# Autodesk Inventor assembly: platform
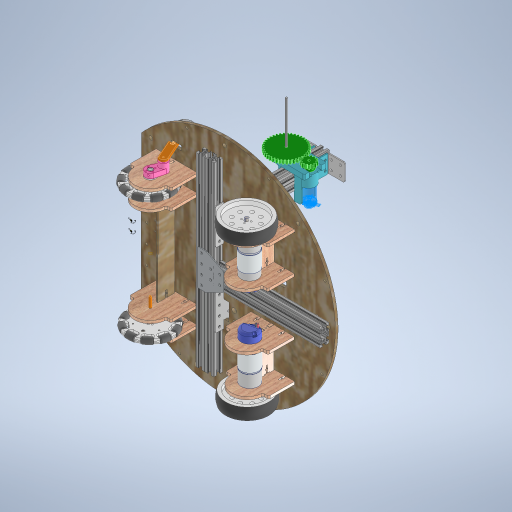
[picture p0: Inventor's stored thumbnail of the model, 512x512]
Saved by Autodesk Inventor 2023.1 (Build 271208000, 208)
## iProperties
Created: 2023-03-13
Part Number: platform
Document SubType Name: Assembly
Designer: User
Author: User
## Documents named in this file (48)
- C:\Users\DELL\reposGitHub\Cheburashka\Cheburashka_construction\platform\platform.iam
- C:\Users\DELL\reposGitHub\Cheburashka\Cheburashka_construction\platform\Osn. platform.ipt
- C:\Users\DELL\reposGitHub\Cheburashka\Cheburashka_construction\platform\motor1.ipt
- C:\Users\DELL\reposGitHub\Cheburashka\Cheburashka_construction\platform\motor2.ipt
- C:\Users\DELL\reposGitHub\Cheburashka\Cheburashka_construction\platform\motor3.ipt
- C:\Users\DELL\reposGitHub\Cheburashka\Cheburashka_construction\platform\wheel1.ipt
- C:\Users\DELL\reposGitHub\Cheburashka\Cheburashka_construction\platform\44260_txm torquenado dc motor_MIR2.ipt
- C:\Users\DELL\reposGitHub\Cheburashka\Cheburashka_construction\platform\36466_txm-4 inch omni wheel.ipt
- C:\Users\DELL\reposGitHub\Cheburashka\Cheburashka_construction\platform\39055_txm-4 inch wheel_MIR1.ipt
- C:\Users\DELL\reposGitHub\Cheburashka\Cheburashka_construction\platform\motor1_MIR3.ipt
- C:\Users\DELL\reposGitHub\Cheburashka\Cheburashka_construction\platform\motor2_MIR3.ipt
- C:\Users\DELL\reposGitHub\Cheburashka\Cheburashka_construction\platform\motor3_MIR3.ipt
- C:\Users\DELL\reposGitHub\Cheburashka\Cheburashka_construction\platform\44260_txm torquenado dc motor_MIR2_MIR.ipt
- C:\Users\DELL\reposGitHub\Cheburashka\Cheburashka_construction\platform\wheel1_MIR.ipt
- C:\Users\DELL\reposGitHub\Cheburashka\Cheburashka_construction\platform\36466_txm-4 inch omni wheel_MIR2.ipt
- C:\Users\DELL\reposGitHub\Cheburashka\Cheburashka_construction\platform\39055_txm-4 inch wheel_MIR1_MIR.ipt
- C:\Users\DELL\reposGitHub\Cheburashka\Cheburashka_construction\platform\кривошип.ipt
- C:\Users\DELL\reposGitHub\Cheburashka\Cheburashka_construction\platform\ось колес2.ipt
- C:\Users\DELL\reposGitHub\Cheburashka\Cheburashka_construction\platform\akfytw2.ipt
- C:\Users\DELL\reposGitHub\Cheburashka\Cheburashka_construction\platform\подшипник2.ipt
- C:\Users\DELL\reposGitHub\Cheburashka\Cheburashka_construction\platform\шатун22.ipt
- C:\Users\DELL\reposGitHub\Cheburashka\Cheburashka_construction\platform\обр_профиль.ipt
- C:\Users\DELL\reposGitHub\Cheburashka\Cheburashka_construction\platform\обр_профиль2.ipt
- C:\Users\DELL\reposGitHub\Cheburashka\Cheburashka_construction\platform\8bc17c1464c21f56fb2a3979b7c6b729.ipt
- C:\Users\DELL\reposGitHub\Cheburashka\Cheburashka_construction\platform\L72-T_soedinitel-60kh80.ipt
- C:\Users\DELL\reposGitHub\Cheburashka\Cheburashka_construction\platform\ребро.ipt
- C:\Users\DELL\reposGitHub\Cheburashka\Cheburashka_construction\platform\стенд.ipt
- C:\Users\DELL\reposGitHub\Cheburashka\Cheburashka_construction\platform\Raspberry Pi Camera Stand - 274111\files\camera_back_cover_v002.ipt
- C:\Users\DELL\reposGitHub\Cheburashka\Cheburashka_construction\platform\Raspberry Pi Camera Stand - 274111\files\camera_front_box_v003.ipt
- C:\Users\DELL\reposGitHub\Cheburashka\Cheburashka_construction\platform\4ad8d019baf454c6bbd45c2c6ffb6783.ipt
- C:\Users\DELL\reposGitHub\Cheburashka\Cheburashka_construction\platform\гриб.ipt
- C:\Users\DELL\reposGitHub\Cheburashka\Cheburashka_construction\platform\legs\myMotorHolder.ipt
- C:\Users\DELL\reposGitHub\Cheburashka\Cheburashka_construction\platform\legs\myBering.ipt
- C:\Users\DELL\reposGitHub\Cheburashka\Cheburashka_construction\platform\legs\POLULU final.ipt
- C:\Users\DELL\reposGitHub\Cheburashka\Cheburashka_construction\platform\legs\axis.ipt
- C:\Users\DELL\reposGitHub\Cheburashka\Cheburashka_construction\platform\legs\bering.ipt
- C:\Users\DELL\reposGitHub\Cheburashka\Cheburashka_construction\platform\8bc17c1464c21f56fb2a3979b7c6b729_MIR.ipt
- C:\Users\DELL\reposGitHub\Cheburashka\Cheburashka_construction\platform\legs\myMotorHolder_MIR.ipt
- C:\Users\DELL\reposGitHub\Cheburashka\Cheburashka_construction\platform\legs\POLULU final_MIR.ipt
- C:\Users\DELL\reposGitHub\Cheburashka\Cheburashka_construction\platform\legs\myBering_MIR.ipt
- C:\Users\DELL\reposGitHub\Cheburashka\Cheburashka_construction\platform\legs\axis_MIR.ipt
- C:\Users\DELL\reposGitHub\Cheburashka\Cheburashka_construction\platform\legs\bering_MIR.ipt
- C:\Users\DELL\reposGitHub\Cheburashka\Cheburashka_construction\platform\legs\шестерня12 (2).ipt
- C:\Users\DELL\reposGitHub\Cheburashka\Cheburashka_construction\platform\legs\шестерня36_v2.ipt
- C:\Users\DELL\reposGitHub\Cheburashka\Cheburashka_construction\platform\legs\шестерня12 (2)_MIR.ipt
- C:\Users\DELL\reposGitHub\Cheburashka\Cheburashka_construction\platform\legs\шестерня36_v2_MIR.ipt
- C:\Users\DELL\reposGitHub\Cheburashka\Cheburashka_construction\platform\8bc17c1464c21f56fb2a3979b7c6b729_MIR1.ipt
- C:\Users\DELL\reposGitHub\Cheburashka\Cheburashka_construction\platform\подш_ноги.ipt
## Components (60 placed, 47 different names)
1. Osn. platform:1 — Совмещение:129, Совмещение:130, Совмещение:131, Совмещение:132, Совмещение:133, Совмещение:137, Совмещение:138, Совмещение:155, Совмещение:158, Совмещение:178, Совмещение:181, Совмещение:182, Совмещение:183, Совмещение:184, Совмещение:185, Совмещение:186, Совмещение:192, Совмещение:193, Совмещение:194, Совмещение:195, Совмещение:196, Совмещение:197, Совмещение:198, Совмещение:217, Совмещение:218, Совмещение:219, Совмещение:230, Совмещение:231, Совмещение:232, Совмещение:233, Совмещение:280, Совмещение:281, Совмещение:282
2. motor1:1 — Совмещение:181, Совмещение:182
3. motor2:1 — Совмещение:232, Совмещение:233
4. motor3:1 — Совмещение:230, Совмещение:231
5. 44260_txm torquenado dc motor_MIR2:1 — Совмещение:21
6. wheel1:1 — Совмещение:101, Совмещение:185, Совмещение:186
7. 36466_txm-4 inch omni wheel:1
8. 39055_txm-4 inch wheel_MIR1:1 — Совмещение:21
9. motor1_MIR3:1 — Совмещение:183, Совмещение:184
10. motor2_MIR3:1 — Совмещение:148
11. motor3_MIR3:1 — Совмещение:109, Совмещение:110, Совмещение:111
12. 44260_txm torquenado dc motor_MIR2_MIR:1 — Совмещение:28, Совмещение:109, Совмещение:110, Совмещение:148
13. wheel1_MIR:1 — Совмещение:192, Совмещение:197, Совмещение:198, Совмещение:228
14. wheel1_MIR:2 — Совмещение:195, Совмещение:196
15. 36466_txm-4 inch omni wheel_MIR2:1 — Совмещение:229
16. 39055_txm-4 inch wheel_MIR1_MIR:1 — Совмещение:28, Совмещение:111
17. кривошип:1 — Совмещение:90, Совмещение:91, Совмещение:92, Совмещение:93, Совмещение:96
18. ось колес2:1 — Совмещение:228, Совмещение:229, Совмещение:283
19. akfytw2:1 — Совмещение:90, Совмещение:91, Совмещение:101, Совмещение:283
20. подшипник2:1 — Совмещение:92, Совмещение:93, Совмещение:94
21. подшипник2:2 — Совмещение:94, Совмещение:95
22. шатун22:1 — Совмещение:95, Совмещение:96, Совмещение:225, Совмещение:226, Совмещение:227
23. обр_профиль:1 — Совмещение:129, Совмещение:130, Совмещение:131, Совмещение:179, Совмещение:206, Совмещение:207, Совмещение:208, Совмещение:210, Симметрия:1
24. обр_профиль:2 — Совмещение:132, Совмещение:133, Совмещение:135, Совмещение:136, Совмещение:157, Совмещение:212, Совмещение:237, Совмещение:238, Совмещение:242, Совмещение:243, Совмещение:250, Совмещение:252, Совмещение:253, Заподлицо:1, Заподлицо:2, Симметрия:1, Совмещение:290
25. обр_профиль2:1 — Совмещение:135, Совмещение:136, Совмещение:139, Совмещение:204, Совмещение:205, Совмещение:209, Совмещение:211
26. обр_профиль:3 — Совмещение:137, Совмещение:138, Совмещение:139
27. 8bc17c1464c21f56fb2a3979b7c6b729:1 — Совмещение:155, Совмещение:206, Совмещение:207
28. 8bc17c1464c21f56fb2a3979b7c6b729:2 — Совмещение:157, Совмещение:158
29. L72-T_soedinitel-60kh80:1 — Совмещение:209, Совмещение:210
30. L72-T_soedinitel-60kh80:2 — Совмещение:211, Совмещение:212
31. L72-T_soedinitel-60kh80:3 — Совмещение:204, Совмещение:205
32. ребро:1 — Совмещение:201, Совмещение:202, Совмещение:203
33. camera_back_cover_v002:1 — Совмещение:222, Совмещение:223, Совмещение:224
34. camera_front_box_v003:1 — Совмещение:220, Совмещение:221, Совмещение:222, Совмещение:223, Совмещение:224
35. 4ad8d019baf454c6bbd45c2c6ffb6783:1 — Совмещение:178, Совмещение:179, Совмещение:208
36. wheel1:2 — Совмещение:193, Совмещение:194, Совмещение:201, Совмещение:202, Совмещение:203
37. стенд:1 — Совмещение:217, Совмещение:218, Совмещение:219, Совмещение:220, Совмещение:221
38. гриб:1 — Совмещение:225, Совмещение:226, Совмещение:227
39. 8bc17c1464c21f56fb2a3979b7c6b729:3 — Совмещение:237, Совмещение:238, Заподлицо:2, Совмещение:291
40. myMotorHolder:1 — Совмещение:247, Совмещение:270, Заподлицо:4, Совмещение:286, Совмещение:289, Совмещение:290, Совмещение:291
41. 8bc17c1464c21f56fb2a3979b7c6b729:4 — Совмещение:242, Совмещение:243, Совмещение:251, Заподлицо:1
42. myBering:1 — Совмещение:250, Совмещение:251, Совмещение:252, Совмещение:253, Совмещение:259
43. POLULU final:1 — Совмещение:247, Совмещение:269
44. axis:1 — Совмещение:287
45. bering:1 — Совмещение:289
46. bering:2 — Совмещение:259
47. 8bc17c1464c21f56fb2a3979b7c6b729_MIR:1 — Совмещение:277, Совмещение:278, Совмещение:279
48. myMotorHolder_MIR:1 — Совмещение:262, Совмещение:263, Совмещение:277, Совмещение:278, Совмещение:279
49. POLULU final_MIR:1 — Совмещение:262, Совмещение:263
50. myBering_MIR:1 — Совмещение:264, Совмещение:265, Совмещение:266, Совмещение:267
51. axis_MIR:1 — Совмещение:264, Совмещение:268
52. bering_MIR:1 — Совмещение:265, Совмещение:266
53. bering_MIR:2 — Совмещение:267, Совмещение:268
54. шестерня12 (2):1 — Совмещение:269, Совмещение:270
55. шестерня36_v2:1 — Совмещение:285, Совмещение:286, Совмещение:287
56. 4ad8d019baf454c6bbd45c2c6ffb6783:2 — Совмещение:280, Совмещение:281, Совмещение:282
57. шестерня12 (2)_MIR:1
58. шестерня36_v2_MIR:1
59. 8bc17c1464c21f56fb2a3979b7c6b729_MIR1:1
60. подш_ноги:1 — Заподлицо:4, Совмещение:285
## Relationships (107: Mate 103, Flush 3, Symmetry 1)
- Совмещение:21 [Mate]: 44260_txm torquenado dc motor_MIR2:1 ↔ 39055_txm-4 inch wheel_MIR1:1
- Совмещение:28 [Mate]: 44260_txm torquenado dc motor_MIR2_MIR:1 ↔ 39055_txm-4 inch wheel_MIR1_MIR:1
- Совмещение:90 [Mate]: кривошип:1 ↔ akfytw2:1
- Совмещение:91 [Mate]: кривошип:1 ↔ akfytw2:1
- Совмещение:92 [Mate]: кривошип:1 ↔ подшипник2:1
- Совмещение:93 [Mate]: кривошип:1 ↔ подшипник2:1
- Совмещение:94 [Mate]: подшипник2:1 ↔ подшипник2:2
- Совмещение:95 [Mate]: подшипник2:2 ↔ шатун22:1
- Совмещение:96 [Mate] (2 mm): кривошип:1 ↔ шатун22:1
- Совмещение:101 [Mate]: wheel1:1 ↔ akfytw2:1
- Совмещение:109 [Mate]: motor3_MIR3:1 ↔ 44260_txm torquenado dc motor_MIR2_MIR:1
- Совмещение:110 [Mate]: motor3_MIR3:1 ↔ 44260_txm torquenado dc motor_MIR2_MIR:1
- Совмещение:111 [Mate] (5 mm): motor3_MIR3:1 ↔ 39055_txm-4 inch wheel_MIR1_MIR:1
- Совмещение:129 [Mate]: Osn. platform:1 ↔ обр_профиль:1
- Совмещение:130 [Mate]: Osn. platform:1 ↔ обр_профиль:1
- Совмещение:131 [Mate]: Osn. platform:1 ↔ обр_профиль:1
- Совмещение:132 [Mate]: Osn. platform:1 ↔ обр_профиль:2
- Совмещение:133 [Mate]: Osn. platform:1 ↔ обр_профиль:2
- Совмещение:135 [Mate] (99.253 mm): обр_профиль:2 ↔ обр_профиль2:1
- Совмещение:136 [Mate]: обр_профиль:2 ↔ обр_профиль2:1
- Совмещение:137 [Mate]: Osn. platform:1 ↔ обр_профиль:3
- Совмещение:138 [Mate] (4.43 mm): Osn. platform:1 ↔ обр_профиль:3
- Совмещение:139 [Mate]: обр_профиль2:1 ↔ обр_профиль:3
- Совмещение:148 [Mate]: motor2_MIR3:1 ↔ 44260_txm torquenado dc motor_MIR2_MIR:1
- Совмещение:155 [Mate]: Osn. platform:1 ↔ 8bc17c1464c21f56fb2a3979b7c6b729:1
- Совмещение:157 [Mate]: обр_профиль:2 ↔ 8bc17c1464c21f56fb2a3979b7c6b729:2
- Совмещение:158 [Mate]: Osn. platform:1 ↔ 8bc17c1464c21f56fb2a3979b7c6b729:2
- Совмещение:178 [Mate]: Osn. platform:1 ↔ 4ad8d019baf454c6bbd45c2c6ffb6783:1
- Совмещение:179 [Mate]: обр_профиль:1 ↔ 4ad8d019baf454c6bbd45c2c6ffb6783:1
- Совмещение:181 [Mate]: Osn. platform:1 ↔ motor1:1
- Совмещение:182 [Mate]: Osn. platform:1 ↔ motor1:1
- Совмещение:183 [Mate]: Osn. platform:1 ↔ motor1_MIR3:1
- Совмещение:184 [Mate]: Osn. platform:1 ↔ motor1_MIR3:1
- Совмещение:185 [Mate]: Osn. platform:1 ↔ wheel1:1
- Совмещение:186 [Mate]: Osn. platform:1 ↔ wheel1:1
- Совмещение:192 [Mate]: Osn. platform:1 ↔ wheel1_MIR:1
- Совмещение:193 [Mate]: Osn. platform:1 ↔ wheel1:2
- Совмещение:194 [Mate]: Osn. platform:1 ↔ wheel1:2
- Совмещение:195 [Mate]: Osn. platform:1 ↔ wheel1_MIR:2
- Совмещение:196 [Mate]: Osn. platform:1 ↔ wheel1_MIR:2
- Совмещение:197 [Mate]: Osn. platform:1 ↔ wheel1_MIR:1
- Совмещение:198 [Mate]: Osn. platform:1 ↔ wheel1_MIR:1
- Совмещение:201 [Mate]: ребро:1 ↔ wheel1:2
- Совмещение:202 [Mate]: ребро:1 ↔ wheel1:2
- Совмещение:203 [Mate]: ребро:1 ↔ wheel1:2
- Совмещение:204 [Mate]: обр_профиль2:1 ↔ L72-T_soedinitel-60kh80:3
- Совмещение:205 [Mate]: обр_профиль2:1 ↔ L72-T_soedinitel-60kh80:3
- Совмещение:206 [Mate]: обр_профиль:1 ↔ 8bc17c1464c21f56fb2a3979b7c6b729:1
- Совмещение:207 [Mate]: обр_профиль:1 ↔ 8bc17c1464c21f56fb2a3979b7c6b729:1
- Совмещение:208 [Mate]: обр_профиль:1 ↔ 4ad8d019baf454c6bbd45c2c6ffb6783:1
- Совмещение:209 [Mate]: обр_профиль2:1 ↔ L72-T_soedinitel-60kh80:1
- Совмещение:210 [Mate]: обр_профиль:1 ↔ L72-T_soedinitel-60kh80:1
- Совмещение:211 [Mate]: обр_профиль2:1 ↔ L72-T_soedinitel-60kh80:2
- Совмещение:212 [Mate]: обр_профиль:2 ↔ L72-T_soedinitel-60kh80:2
- Совмещение:217 [Mate]: Osn. platform:1 ↔ стенд:1
- Совмещение:218 [Mate]: Osn. platform:1 ↔ стенд:1
- Совмещение:219 [Mate]: Osn. platform:1 ↔ стенд:1
- Совмещение:220 [Mate]: camera_front_box_v003:1 ↔ стенд:1
- Совмещение:221 [Mate]: camera_front_box_v003:1 ↔ стенд:1
- Совмещение:222 [Mate]: camera_back_cover_v002:1 ↔ camera_front_box_v003:1
- Совмещение:223 [Mate]: camera_back_cover_v002:1 ↔ camera_front_box_v003:1
- Совмещение:224 [Mate]: camera_back_cover_v002:1 ↔ camera_front_box_v003:1
- Совмещение:225 [Mate]: шатун22:1 ↔ гриб:1
- Совмещение:226 [Mate]: шатун22:1 ↔ гриб:1
- Совмещение:227 [Mate] (-1.6 mm): шатун22:1 ↔ гриб:1
- Совмещение:228 [Mate]: wheel1_MIR:1 ↔ ось колес2:1
- Совмещение:229 [Mate]: 36466_txm-4 inch omni wheel_MIR2:1 ↔ ось колес2:1
- Совмещение:230 [Mate]: Osn. platform:1 ↔ motor3:1
- Совмещение:231 [Mate]: Osn. platform:1 ↔ motor3:1
- Совмещение:232 [Mate]: Osn. platform:1 ↔ motor2:1
- Совмещение:233 [Mate]: Osn. platform:1 ↔ motor2:1
- Совмещение:237 [Mate]: обр_профиль:2 ↔ 8bc17c1464c21f56fb2a3979b7c6b729:3
- Совмещение:238 [Mate]: обр_профиль:2 ↔ 8bc17c1464c21f56fb2a3979b7c6b729:3
- Совмещение:242 [Mate]: обр_профиль:2 ↔ 8bc17c1464c21f56fb2a3979b7c6b729:4
- Совмещение:243 [Mate]: обр_профиль:2 ↔ 8bc17c1464c21f56fb2a3979b7c6b729:4
- Совмещение:247 [Mate]: myMotorHolder:1 ↔ POLULU final:1
- Совмещение:250 [Mate]: обр_профиль:2 ↔ myBering:1
- Совмещение:251 [Mate]: 8bc17c1464c21f56fb2a3979b7c6b729:4 ↔ myBering:1
- Совмещение:252 [Mate]: обр_профиль:2 ↔ myBering:1
- Совмещение:253 [Mate]: обр_профиль:2 ↔ myBering:1
- Совмещение:259 [Mate]: myBering:1 ↔ bering:2
- Заподлицо:1 [Flush] (4 mm): обр_профиль:2 ↔ 8bc17c1464c21f56fb2a3979b7c6b729:4
- Заподлицо:2 [Flush] (4 mm): обр_профиль:2 ↔ 8bc17c1464c21f56fb2a3979b7c6b729:3
- Симметрия:1 [Symmetry]: обр_профиль:1 ↔ обр_профиль:2
- Совмещение:262 [Mate]: myMotorHolder_MIR:1 ↔ POLULU final_MIR:1
- Совмещение:263 [Mate]: myMotorHolder_MIR:1 ↔ POLULU final_MIR:1
- Совмещение:264 [Mate]: myBering_MIR:1 ↔ axis_MIR:1
- Совмещение:265 [Mate]: myBering_MIR:1 ↔ bering_MIR:1
- Совмещение:266 [Mate]: myBering_MIR:1 ↔ bering_MIR:1
- Совмещение:267 [Mate]: myBering_MIR:1 ↔ bering_MIR:2
- Совмещение:268 [Mate]: axis_MIR:1 ↔ bering_MIR:2
- Совмещение:269 [Mate]: POLULU final:1 ↔ шестерня12 (2):1
- Совмещение:270 [Mate] (2 mm): myMotorHolder:1 ↔ шестерня12 (2):1
- Совмещение:277 [Mate]: 8bc17c1464c21f56fb2a3979b7c6b729_MIR:1 ↔ myMotorHolder_MIR:1
- Совмещение:278 [Mate]: 8bc17c1464c21f56fb2a3979b7c6b729_MIR:1 ↔ myMotorHolder_MIR:1
- Совмещение:279 [Mate]: 8bc17c1464c21f56fb2a3979b7c6b729_MIR:1 ↔ myMotorHolder_MIR:1
- Совмещение:280 [Mate]: Osn. platform:1 ↔ 4ad8d019baf454c6bbd45c2c6ffb6783:2
- Совмещение:281 [Mate]: Osn. platform:1 ↔ 4ad8d019baf454c6bbd45c2c6ffb6783:2
- Совмещение:282 [Mate]: Osn. platform:1 ↔ 4ad8d019baf454c6bbd45c2c6ffb6783:2
- Совмещение:283 [Mate]: ось колес2:1 ↔ akfytw2:1
- Заподлицо:4 [Flush]: myMotorHolder:1 ↔ подш_ноги:1
- Совмещение:285 [Mate]: шестерня36_v2:1 ↔ подш_ноги:1
- Совмещение:286 [Mate] (1 mm): myMotorHolder:1 ↔ шестерня36_v2:1
- Совмещение:287 [Mate]: axis:1 ↔ шестерня36_v2:1
- Совмещение:289 [Mate]: myMotorHolder:1 ↔ bering:1
- Совмещение:290 [Mate]: обр_профиль:2 ↔ myMotorHolder:1
- Совмещение:291 [Mate]: 8bc17c1464c21f56fb2a3979b7c6b729:3 ↔ myMotorHolder:1
